# Autodesk Inventor assembly: west coast drive base
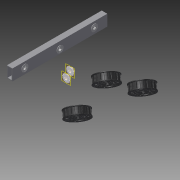
[picture p0: Inventor's stored thumbnail of the model, 180x180]
Saved by Autodesk Inventor 2013 (Build 170138000, 138)
## iProperties
Created: 2014-07-12
Part Number: west coast drive base
Document SubType Name: Assembly
Designer: admin
Author: admin
## Documents named in this file (5)
- C:\Users\admin\Documents\GitHub\CAD\west coast drive\west coast drive base.iam
- C:\Users\admin\Documents\GitHub\2013-2014_BlockParty\CAD\COTSParts\Sprockets - AndyMark\25 sprocket 16T 500Hex.ipt
- C:\Users\admin\Documents\GitHub\2013-2014_BlockParty\CAD\COTSParts\Bearings - VexPro\Flanged Bearing - 0.5in Hex ID x 1.125in OD.ipt
- C:\Users\admin\Documents\GitHub\CAD\west coast drive\side 1.ipt
- C:\Users\admin\Documents\GitHub\CAD\west coast drive\Wheel Vexpro 4in .iam
## Components (12 placed, 4 different names)
1. Roller Chain Sprocket2:1
2. Roller Chain Sprocket2:2
3. Flanged Bearing - 0.5in Hex ID x 1.125in OD:1 — Mate:13, Mate:14, Flush:1
4. Flanged Bearing - 0.5in Hex ID x 1.125in OD:2 — Mate:11, Mate:12, Flush:1
5. side 1:1 — Mate:11, Mate:12, Mate:13, Mate:14, Mate:15, Mate:16, Mate:17, Mate:18, Mate:19, Mate:20, Mate:21, Mate:22
6. Wheel Vexpro 4in :1 [sub-assembly]
7. Wheel Vexpro 4in :2 [sub-assembly]
8. Wheel Vexpro 4in :3 [sub-assembly]
9. Flanged Bearing - 0.5in Hex ID x 1.125in OD:3 — Mate:17, Mate:19
10. Flanged Bearing - 0.5in Hex ID x 1.125in OD:4 — Mate:18, Mate:21
11. Flanged Bearing - 0.5in Hex ID x 1.125in OD:5 — Mate:15, Mate:16
12. Flanged Bearing - 0.5in Hex ID x 1.125in OD:6 — Mate:20, Mate:22
## Relationships (13: Mate 12, Flush 1)
- Mate:11: Flanged Bearing - 0.5in Hex ID x 1.125in OD:2 ↔ side 1:1
- Mate:12: Flanged Bearing - 0.5in Hex ID x 1.125in OD:2 ↔ side 1:1
- Mate:13: Flanged Bearing - 0.5in Hex ID x 1.125in OD:1 ↔ side 1:1
- Mate:14: Flanged Bearing - 0.5in Hex ID x 1.125in OD:1 ↔ side 1:1
- Flush:1: Flanged Bearing - 0.5in Hex ID x 1.125in OD:1 ↔ Flanged Bearing - 0.5in Hex ID x 1.125in OD:2
- Mate:15: side 1:1 ↔ Flanged Bearing - 0.5in Hex ID x 1.125in OD:5
- Mate:16: side 1:1 ↔ Flanged Bearing - 0.5in Hex ID x 1.125in OD:5
- Mate:17: side 1:1 ↔ Flanged Bearing - 0.5in Hex ID x 1.125in OD:3
- Mate:18: side 1:1 ↔ Flanged Bearing - 0.5in Hex ID x 1.125in OD:4
- Mate:19: side 1:1 ↔ Flanged Bearing - 0.5in Hex ID x 1.125in OD:3
- Mate:20: side 1:1 ↔ Flanged Bearing - 0.5in Hex ID x 1.125in OD:6
- Mate:21: side 1:1 ↔ Flanged Bearing - 0.5in Hex ID x 1.125in OD:4
- Mate:22: side 1:1 ↔ Flanged Bearing - 0.5in Hex ID x 1.125in OD:6
